# Autodesk Inventor assembly: ProbeHead V2 - Assembly
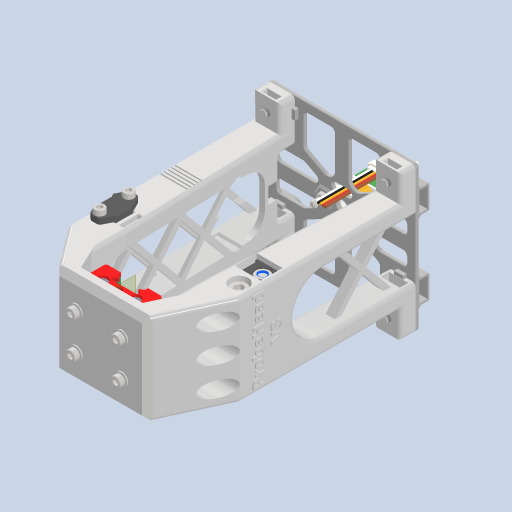
[picture p0: Inventor's stored thumbnail of the model, 512x512]
Saved by Autodesk Inventor 2023.2 (Build 272271000, 271)
## iProperties
Created: 2024-02-09
Part Number: ProbeHead V2 - Assembly
Document SubType Name: Assembly
Designer: Nils Bade
Author: Nils Bade
## Documents named in this file (16)
- C:\Users\nilsb\Documents\Inventor\Projektarbeit-Bade\RatRig_modified\ProbeHead\LevelingHead V1 - Assembly.iam
- C:\Users\nilsb\Documents\Inventor\Projektarbeit-Bade\RatRig_Standards\core_xy_belt_grabber v2.ipt
- C:\Users\nilsb\Documents\Inventor\Projektarbeit-Bade\RatRig_modified\MGN15 Linear-Rail-Block.ipt
- C:\Users\nilsb\Documents\Inventor\Projektarbeit-Bade\RatRig_Standards\face_belt_grabber v2.ipt
- C:\Users\nilsb\Documents\Inventor\Projektarbeit-Bade\Schrauben\Cap Head Screw M3x12 v2.ipt
- C:\Users\nilsb\Documents\Inventor\Projektarbeit-Bade\RatRig_Standards\Hex Nut - M3 v2.ipt
- C:\Users\nilsb\Documents\Inventor\Projektarbeit-Bade\Schrauben\Cap Head Screw M5x40 v2.ipt
- C:\Users\nilsb\Documents\Inventor\Projektarbeit-Bade\RatRig_Standards\Hex Locking Nut - M5 v2.ipt
- C:\Users\nilsb\Documents\Inventor\Projektarbeit-Bade\Schrauben\Cap Head Screw M4x12 - DIN912.ipt
- C:\Users\nilsb\Documents\Inventor\Projektarbeit-Bade\Schrauben\Washer Simple M3 - DIN6902.ipt
- C:\Users\nilsb\Documents\Inventor\Projektarbeit-Bade\RatRig_modified\ProbeHead\BLTouch Sensor V3_1.ipt
- BL Touch Sensor.ipt
- C:\Users\nilsb\Documents\Inventor\Projektarbeit-Bade\RatRig_Standards\Hex Locking Nut - M3 v2.ipt
- C:\Users\nilsb\Documents\Inventor\Projektarbeit-Bade\RatRig_Standards\Hex Nut - M4 DIN934.ipt
- C:\Users\nilsb\Documents\Inventor\Projektarbeit-Bade\RatRig_modified\ProbeHead\ProbeHead-Arms V3.ipt
- C:\Users\nilsb\Documents\Inventor\Projektarbeit-Bade\RatRig_modified\ProbeHead\BLTouch-Leveling-Plate_V2.ipt
## Components (40 placed, 14 different names)
1. ProbeHead-Arms_V3:1 — Passend:76, Passend:77, Passend:78, Passend:79, Winkel:18, Winkel:19, Winkel:20, Winkel:21, Passend:80, Passend:81, Passend:82, Passend:83, Passend:90, Passend:91
2. core_xy_belt_grabber v2:1 — Winkel:7, Passend:35
3. core_xy_belt_grabber v2:2 — Passend:32, Passend:33, Winkel:8
4. MGN15 Linear-Rail-Block:1
5. face_belt_grabber v2:1 — Passend:16, Passend:17, Passend:18, Passend:19
6. face_belt_grabber v2:2 — Passend:12, Passend:13, Passend:14, Passend:15
7. Cap Head Screw M3x12 v2:1 — Passend:16, Passend:18, Passend:20
8. Cap Head Screw M3x12 v2:2 — Passend:17, Passend:19, Passend:21
9. Cap Head Screw M3x12 v2:3 — Passend:12, Passend:14, Passend:22
10. Cap Head Screw M3x12 v2:4 — Passend:13, Passend:15, Passend:23
11. Hex Nut - M3 v2:1 — Passend:20
12. Hex Nut - M3 v2:2 — Passend:23
13. Hex Nut - M3 v2:3 — Passend:22
14. Hex Nut - M3 v2:4 — Passend:21
15. Cap Head Screw M5x40 v2:1 — Passend:34
16. Cap Head Screw M5x40 v2:2
17. Hex Locking Nut - M5 v2:1 — Passend:32, Passend:33, Winkel:8
18. Hex Locking Nut - M5 v2:2 — Passend:34, Winkel:7, Passend:35
19. Cap Head Screw M4x12 - DIN912:1 — Passend:93, Passend:98
20. Cap Head Screw M4x12 - DIN912:2 — Passend:94, Passend:99
21. Cap Head Screw M4x12 - DIN912:3 — Passend:92, Passend:97
22. Cap Head Screw M4x12 - DIN912:4 — Passend:95, Passend:96
23. Washer Simple M3 - DIN6902:1 — Passend:59
24. Washer Simple M3 - DIN6902:2 — Passend:56
25. Washer Simple M3 - DIN6902:3 — Passend:58
26. Washer Simple M3 - DIN6902:4 — Passend:57
27. Cap Head Screw M3x12 v2:5 — Passend:59
28. Cap Head Screw M3x12 v2:6 — Passend:58
29. Cap Head Screw M3x12 v2:7 — Passend:56
30. Cap Head Screw M3x12 v2:8 — Passend:57
31. BLTouch-Leveling-Plate_V2:1 — Passend:84, Passend:85, Winkel:22, Winkel:23, Passend:88, Passend:89, Passend:90, Passend:91, Passend:92, Passend:93, Passend:94, Passend:95, Passend:96, Passend:97, Passend:98, Passend:99
32. BL Touch Sensor:1 — Passend:72, Passend:73, Passend:74, Passend:75
33. Hex Locking Nut - M3 v2:1 — Passend:87, Winkel:22, Passend:88
34. Hex Locking Nut - M3 v2:2 — Passend:86, Winkel:23, Passend:89
35. Cap Head Screw M3x12 v2:9 — Passend:72, Passend:75, Passend:85, Passend:86
36. Cap Head Screw M3x12 v2:10 — Passend:73, Passend:74, Passend:84, Passend:87
37. Hex Nut - M4 DIN934:1 — Passend:78, Winkel:18, Passend:82
38. Hex Nut - M4 DIN934:2 — Passend:77, Winkel:20, Passend:81
39. Hex Nut - M4 DIN934:3 — Passend:79, Winkel:19, Passend:83
40. Hex Nut - M4 DIN934:4 — Passend:76, Winkel:21, Passend:80
## Relationships (97: Mate 81, Angle 14, Flush 2)
- [Mate]: ProbeHead-Arms_V3:1 ↔ MGN15 Linear-Rail-Block:1
- [Mate]: ProbeHead-Arms_V3:1 ↔ MGN15 Linear-Rail-Block:1
- [Mate]: ProbeHead-Arms_V3:1 ↔ MGN15 Linear-Rail-Block:1
- [Mate]: ProbeHead-Arms_V3:1 ↔ core_xy_belt_grabber v2:2
- [Angle] (0 deg): ProbeHead-Arms_V3:1 ↔ core_xy_belt_grabber v2:1
- [Mate]: ProbeHead-Arms_V3:1 ↔ core_xy_belt_grabber v2:1
- [Flush] (2 mm): ProbeHead-Arms_V3:1 ↔ core_xy_belt_grabber v2:1
- [Flush] (2 mm): ProbeHead-Arms_V3:1 ↔ core_xy_belt_grabber v2:2
- [Mate]: ProbeHead-Arms_V3:1 ↔ face_belt_grabber v2:2
- [Mate]: ProbeHead-Arms_V3:1 ↔ face_belt_grabber v2:2
- [Mate]: ProbeHead-Arms_V3:1 ↔ face_belt_grabber v2:1
- [Mate]: ProbeHead-Arms_V3:1 ↔ face_belt_grabber v2:1
- Passend:12 [Mate]: face_belt_grabber v2:2 ↔ Cap Head Screw M3x12 v2:3
- Passend:13 [Mate]: face_belt_grabber v2:2 ↔ Cap Head Screw M3x12 v2:4
- Passend:14 [Mate]: face_belt_grabber v2:2 ↔ Cap Head Screw M3x12 v2:3
- Passend:15 [Mate]: face_belt_grabber v2:2 ↔ Cap Head Screw M3x12 v2:4
- Passend:16 [Mate]: face_belt_grabber v2:1 ↔ Cap Head Screw M3x12 v2:1
- Passend:17 [Mate]: face_belt_grabber v2:1 ↔ Cap Head Screw M3x12 v2:2
- Passend:18 [Mate]: face_belt_grabber v2:1 ↔ Cap Head Screw M3x12 v2:1
- Passend:19 [Mate]: face_belt_grabber v2:1 ↔ Cap Head Screw M3x12 v2:2
- Passend:20 [Mate]: Cap Head Screw M3x12 v2:1 ↔ Hex Nut - M3 v2:1
- Passend:21 [Mate]: Cap Head Screw M3x12 v2:2 ↔ Hex Nut - M3 v2:4
- Passend:22 [Mate]: Cap Head Screw M3x12 v2:3 ↔ Hex Nut - M3 v2:3
- Passend:23 [Mate]: Cap Head Screw M3x12 v2:4 ↔ Hex Nut - M3 v2:2
- [Angle] (0 deg): ProbeHead-Arms_V3:1 ↔ Hex Nut - M3 v2:1
- [Angle] (0 deg): ProbeHead-Arms_V3:1 ↔ Hex Nut - M3 v2:3
- [Mate]: ProbeHead-Arms_V3:1 ↔ Hex Nut - M3 v2:3
- [Mate]: ProbeHead-Arms_V3:1 ↔ Hex Nut - M3 v2:2
- [Mate]: ProbeHead-Arms_V3:1 ↔ Hex Nut - M3 v2:1
- [Mate]: ProbeHead-Arms_V3:1 ↔ Hex Nut - M3 v2:4
- [Mate]: ProbeHead-Arms_V3:1 ↔ Cap Head Screw M5x40 v2:2
- [Mate]: ProbeHead-Arms_V3:1 ↔ Cap Head Screw M5x40 v2:1
- [Mate]: ProbeHead-Arms_V3:1 ↔ Cap Head Screw M5x40 v2:1
- [Mate]: ProbeHead-Arms_V3:1 ↔ Cap Head Screw M5x40 v2:2
- Passend:32 [Mate]: core_xy_belt_grabber v2:2 ↔ Hex Locking Nut - M5 v2:1
- Passend:33 [Mate]: core_xy_belt_grabber v2:2 ↔ Hex Locking Nut - M5 v2:1
- Passend:34 [Mate]: Cap Head Screw M5x40 v2:1 ↔ Hex Locking Nut - M5 v2:2
- Winkel:7 [Angle] (0 deg): core_xy_belt_grabber v2:1 ↔ Hex Locking Nut - M5 v2:2
- Passend:35 [Mate]: core_xy_belt_grabber v2:1 ↔ Hex Locking Nut - M5 v2:2
- Winkel:8 [Angle] (0 deg): core_xy_belt_grabber v2:2 ↔ Hex Locking Nut - M5 v2:1
- [Mate]: ProbeHead-Arms_V3:1 ↔ Washer Simple M3 - DIN6902:1
- [Mate]: ProbeHead-Arms_V3:1 ↔ Washer Simple M3 - DIN6902:2
- [Mate]: ProbeHead-Arms_V3:1 ↔ Washer Simple M3 - DIN6902:3
- [Mate]: ProbeHead-Arms_V3:1 ↔ Washer Simple M3 - DIN6902:4
- [Mate]: ProbeHead-Arms_V3:1 ↔ Washer Simple M3 - DIN6902:4
- [Mate]: ProbeHead-Arms_V3:1 ↔ Washer Simple M3 - DIN6902:2
- [Mate]: ProbeHead-Arms_V3:1 ↔ Washer Simple M3 - DIN6902:1
- [Mate]: ProbeHead-Arms_V3:1 ↔ Washer Simple M3 - DIN6902:3
- [Mate]: ProbeHead-Arms_V3:1 ↔ Cap Head Screw M3x12 v2:5
- [Mate]: ProbeHead-Arms_V3:1 ↔ Cap Head Screw M3x12 v2:6
- [Mate]: ProbeHead-Arms_V3:1 ↔ Cap Head Screw M3x12 v2:7
- [Mate]: ProbeHead-Arms_V3:1 ↔ Cap Head Screw M3x12 v2:8
- Passend:56 [Mate]: Washer Simple M3 - DIN6902:2 ↔ Cap Head Screw M3x12 v2:7
- Passend:57 [Mate]: Washer Simple M3 - DIN6902:4 ↔ Cap Head Screw M3x12 v2:8
- Passend:58 [Mate]: Washer Simple M3 - DIN6902:3 ↔ Cap Head Screw M3x12 v2:6
- Passend:59 [Mate]: Washer Simple M3 - DIN6902:1 ↔ Cap Head Screw M3x12 v2:5
- [Mate]: ProbeHead-Arms_V3:1 ↔ Cap Head Screw M3x12 v2:4
- [Mate]: ProbeHead-Arms_V3:1 ↔ Cap Head Screw M3x12 v2:2
- [Angle] (0 deg): ProbeHead-Arms_V3:1 ↔ Hex Nut - M3 v2:2
- [Angle] (0 deg): ProbeHead-Arms_V3:1 ↔ Hex Nut - M3 v2:4
- [Mate]: ProbeHead-Arms_V3:1 ↔ BLTouch-Leveling-Plate_V2:1
- [Mate]: BLTouch-Leveling-Plate_V2:1 ↔ BL Touch Sensor:1
- Passend:72 [Mate]: BL Touch Sensor:1 ↔ Cap Head Screw M3x12 v2:9
- Passend:73 [Mate]: BL Touch Sensor:1 ↔ Cap Head Screw M3x12 v2:10
- Passend:74 [Mate]: BL Touch Sensor:1 ↔ Cap Head Screw M3x12 v2:10
- Passend:75 [Mate]: BL Touch Sensor:1 ↔ Cap Head Screw M3x12 v2:9
- [Angle] (180 deg): ProbeHead-Arms_V3:1 ↔ core_xy_belt_grabber v2:2
- Passend:76 [Mate]: ProbeHead-Arms_V3:1 ↔ Hex Nut - M4 DIN934:4
- Passend:77 [Mate]: ProbeHead-Arms_V3:1 ↔ Hex Nut - M4 DIN934:2
- Passend:78 [Mate]: ProbeHead-Arms_V3:1 ↔ Hex Nut - M4 DIN934:1
- Passend:79 [Mate]: ProbeHead-Arms_V3:1 ↔ Hex Nut - M4 DIN934:3
- Winkel:18 [Angle] (0 deg): ProbeHead-Arms_V3:1 ↔ Hex Nut - M4 DIN934:1
- Winkel:19 [Angle] (0 deg): ProbeHead-Arms_V3:1 ↔ Hex Nut - M4 DIN934:3
- Winkel:20 [Angle] (0 deg): ProbeHead-Arms_V3:1 ↔ Hex Nut - M4 DIN934:2
- Winkel:21 [Angle] (0 deg): ProbeHead-Arms_V3:1 ↔ Hex Nut - M4 DIN934:4
- Passend:80 [Mate]: ProbeHead-Arms_V3:1 ↔ Hex Nut - M4 DIN934:4
- Passend:81 [Mate]: ProbeHead-Arms_V3:1 ↔ Hex Nut - M4 DIN934:2
- Passend:82 [Mate]: ProbeHead-Arms_V3:1 ↔ Hex Nut - M4 DIN934:1
- Passend:83 [Mate]: ProbeHead-Arms_V3:1 ↔ Hex Nut - M4 DIN934:3
- Passend:84 [Mate]: BLTouch-Leveling-Plate_V2:1 ↔ Cap Head Screw M3x12 v2:10
- Passend:85 [Mate]: BLTouch-Leveling-Plate_V2:1 ↔ Cap Head Screw M3x12 v2:9
- Passend:86 [Mate]: Hex Locking Nut - M3 v2:2 ↔ Cap Head Screw M3x12 v2:9
- Passend:87 [Mate]: Hex Locking Nut - M3 v2:1 ↔ Cap Head Screw M3x12 v2:10
- Winkel:22 [Angle] (0 deg): BLTouch-Leveling-Plate_V2:1 ↔ Hex Locking Nut - M3 v2:1
- Winkel:23 [Angle] (0 deg): BLTouch-Leveling-Plate_V2:1 ↔ Hex Locking Nut - M3 v2:2
- Passend:88 [Mate]: BLTouch-Leveling-Plate_V2:1 ↔ Hex Locking Nut - M3 v2:1
- Passend:89 [Mate]: BLTouch-Leveling-Plate_V2:1 ↔ Hex Locking Nut - M3 v2:2
- Passend:90 [Mate]: ProbeHead-Arms_V3:1 ↔ BLTouch-Leveling-Plate_V2:1
- Passend:91 [Mate]: ProbeHead-Arms_V3:1 ↔ BLTouch-Leveling-Plate_V2:1
- Passend:92 [Mate]: Cap Head Screw M4x12 - DIN912:3 ↔ BLTouch-Leveling-Plate_V2:1
- Passend:93 [Mate]: Cap Head Screw M4x12 - DIN912:1 ↔ BLTouch-Leveling-Plate_V2:1
- Passend:94 [Mate]: Cap Head Screw M4x12 - DIN912:2 ↔ BLTouch-Leveling-Plate_V2:1
- Passend:95 [Mate]: Cap Head Screw M4x12 - DIN912:4 ↔ BLTouch-Leveling-Plate_V2:1
- Passend:96 [Mate]: Cap Head Screw M4x12 - DIN912:4 ↔ BLTouch-Leveling-Plate_V2:1
- Passend:97 [Mate]: Cap Head Screw M4x12 - DIN912:3 ↔ BLTouch-Leveling-Plate_V2:1
- Passend:98 [Mate]: Cap Head Screw M4x12 - DIN912:1 ↔ BLTouch-Leveling-Plate_V2:1
- Passend:99 [Mate]: Cap Head Screw M4x12 - DIN912:2 ↔ BLTouch-Leveling-Plate_V2:1
